# Autodesk Inventor assembly: HexShaft+Toughbox-mini
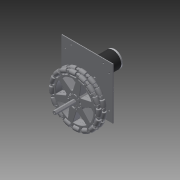
[picture p0: Inventor's stored thumbnail of the model, 180x180]
Saved by Autodesk Inventor 2013 (Build 170138000, 138)
## iProperties
Created: 2013-01-11
Part Number: HexShaft+Toughbox-mini
Document SubType Name: Assembly
Designer: Naphat
Translation Standard: STEP AP203
FileName: S:/Products/Gearboxes Spur Single Stage/Toughbox/Toughbox Mini/Toughbox-Mini.stp
PreProcessor: Unknown
PostProcessor: Build: 138, Release: 2013 RTM - Date: Thu 03/01/2012
Sent Units: millimeter
Uncertainty: 0.001
Author: Naphat
## Documents named in this file (17)
- C:\Users\carneeki\Google Drive\FRC Games\FRC2013\FRC2013 - LDU\Kiwi Robot\HexShaft+Toughbox-mini.iam
- C:\Users\carneeki\Google Drive\FRC Games\FRC2013\FRC2013 - LDU\Kiwi Robot\Toughbox-mini\r6zz.ipt
- C:\Users\carneeki\Google Drive\FRC Games\FRC2013\FRC2013 - LDU\Kiwi Robot\Toughbox-mini\Toughbox_d07.ipt
- C:\Users\carneeki\Google Drive\FRC Games\FRC2013\FRC2013 - LDU\Kiwi Robot\Toughbox-mini\Toughbox_d05.ipt
- C:\Users\carneeki\Google Drive\FRC Games\FRC2013\FRC2013 - LDU\Kiwi Robot\Toughbox-mini\Toughbox_d08.ipt
- C:\Users\carneeki\Google Drive\FRC Games\FRC2013\FRC2013 - LDU\Kiwi Robot\Toughbox-mini\Toughbox_d06.ipt
- C:\Users\carneeki\Google Drive\FRC Games\FRC2013\FRC2013 - LDU\Kiwi Robot\Toughbox-mini\fr-6-zz.ipt
- C:\Users\carneeki\Google Drive\FRC Games\FRC2013\FRC2013 - LDU\Kiwi Robot\Toughbox-mini\fr-8-zz.ipt
- C:\Users\carneeki\Google Drive\FRC Games\FRC2013\FRC2013 - LDU\Kiwi Robot\Toughbox-mini\10-32_nylock_nut.ipt
- C:\Users\carneeki\Google Drive\FRC Games\FRC2013\FRC2013 - LDU\Kiwi Robot\Toughbox-mini\5-16_washer.ipt
- C:\Users\carneeki\Google Drive\FRC Games\FRC2013\FRC2013 - LDU\Kiwi Robot\Toughbox-mini\Toughbox_d09.ipt
- C:\Users\carneeki\Google Drive\FRC Games\FRC2013\FRC2013 - LDU\Kiwi Robot\Toughbox-mini\8mm_spring_clip.ipt
- C:\Users\carneeki\Google Drive\FRC Games\FRC2013\FRC2013 - LDU\Kiwi Robot\Toughbox-mini\Toughbox-mini_d01-5-12.ipt
- C:\Users\carneeki\Google Drive\FRC Games\FRC2013\FRC2013 - LDU\Kiwi Robot\Toughbox-mini\10-32x0625_shcs.ipt
- C:\Users\carneeki\Google Drive\Robotics\FRC 2013\FRC2013 - LDU\Kiwi Robot\Custom GearBox Mount.ipt
- C:\Users\carneeki\Google Drive\FRC Games\FRC2013\FRC2013 - LDU\Kiwi Robot\Vex Wheel\Vex Wheel Assembly.iam
- C:\Users\carneeki\Google Drive\Robotics\FRC 2013\FRC2013 - LDU\Kiwi Robot\Imported Components\Motors\CIM\CIM Motor.iam
## Components (32 placed, 16 different names)
1. r6zz:1
2. r6zz:2 — Insert:1
3. Toughbox_d07:1
4. Toughbox_d05:1
5. Toughbox_d08:1
6. Toughbox_d06:1
7. fr-6-zz:1
8. fr-8-zz:1 — Mate:8
9. 10-32_nylock_nut:1
10. 10-32_nylock_nut:2
11. 10-32_nylock_nut:3
12. 10-32_nylock_nut:4
13. 5-16_washer:1
14. 5-16_washer:2
15. 5-16_washer:3
16. 5-16_washer:4
17. Toughbox_d09:1
18. Toughbox_d09:2
19. 8mm_spring_clip:1
20. 8mm_spring_clip:2
21. Toughbox-mini_d01-5-12:1 — Mate:7
22. 10-32x0625_shcs:1
23. 10-32x0625_shcs:2
24. 10-32x0625_shcs:3
25. 10-32x0625_shcs:4
26. 10-32x0625_shcs:5
27. 10-32x0625_shcs:6
28. 10-32x0625_shcs:7
29. 10-32x0625_shcs:8
30. Custom GearBox Mount:1 — Mate:7, Mate:8, Insert:2
31. Vex Wheel Assembly:1 [sub-assembly] — Insert:1
32. CIM Motor:1 [sub-assembly] — Insert:2
## Relationships (4: Mate 2, Insert 2)
- Mate:7: Toughbox-mini_d01-5-12:1 ↔ Custom GearBox Mount:1
- Mate:8: fr-8-zz:1 ↔ Custom GearBox Mount:1
- Insert:1: r6zz:2 ↔ Vex Wheel Assembly:1
- Insert:2: Custom GearBox Mount:1 ↔ CIM Motor:1
